# Autodesk Inventor assembly: Zylinder_bumper
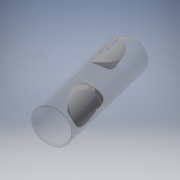
[picture p0: Inventor's stored thumbnail of the model, 180x180]
Saved by Autodesk Inventor 2017 (Build 210142000, 142)
## iProperties
Part Number: Zylinder_bumper
Material: Generisch
Document SubType Name: Assembly
Designer: Fabio
Author: Fabio
## Documents named in this file (3)
- C:\Users\Fabio\dicer\inventor\Zylinder_bumper.iam
- C:\Users\Fabio\dicer\inventor\cylinder.ipt
- C:\Users\Fabio\dicer\inventor\bumper.ipt
## Components (4 placed, 2 different names)
1. cylinder:1 — Passend:1, Passend:3, Passend:4
2. bumper:1 — Passend:3
3. bumper:2 — Passend:1
4. bumper:4 — Passend:4
## Relationships (3: Mate 3)
- Passend:1 [Mate]: cylinder:1 ↔ bumper:2
- Passend:3 [Mate]: cylinder:1 ↔ bumper:1
- Passend:4 [Mate]: cylinder:1 ↔ bumper:4
